# Autodesk Inventor assembly: Elevator Motor Assembly_MIR1 (nano)
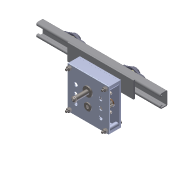
[picture p0: Inventor's stored thumbnail of the model, 180x180]
Saved by Autodesk Inventor 2015 (Build 190159000, 159)
## iProperties
Created: 2015-01-24
Part Number: Elevator Motor Assembly_MIR1 (nano)
Document SubType Name: Assembly
Designer: Peter
Author: Peter
## Documents named in this file (5)
- C:\Users\Tanner\Documents\GitHub\FIRST-Team-1719-CAD-Team\2015 Robot CAD\Lifter Super Structure\Tower\Elevator Motor Assembly\Elevator Motor Assembly_MIR1 (nano).iam
- C:\Users\Tanner\Documents\GitHub\FIRST-Team-1719-CAD-Team\2015 Robot CAD\Lifter Super Structure\Tower\Elevator Motor Assembly\Lower Motor Mount_MIR1.ipt
- C:\Users\Tanner\Documents\GitHub\FIRST-Team-1719-CAD-Team\2015 Robot CAD\Lifter Super Structure\Tower\Elevator Motor Assembly\Andy Mark Tough Box_MIR1.iam
- C:\Users\Tanner\Documents\GitHub\FIRST-Team-1719-CAD-Team\2015 Robot CAD\Lifter Super Structure\Tower\Elevator Motor Assembly\Horizontal-Unistrut-Tower-Connector-15_MIR1.ipt
- C:\Users\Tanner\Documents\GitHub\FIRST-Team-1719-CAD-Team\2015 Robot CAD\Lifter Super Structure\Tower\Elevator Motor Assembly\IGUS EF01-10\EFOI_10_1.iam
## Components (5 placed, 4 different names)
1. Lower Motor Mount_MIR1:1 — Mate:3, Mate:2, Mate:1, Mate:4, Flush:1
2. Andy Mark Tough Box_MIR1:1 [sub-assembly] — Mate:3, Mate:2, Mate:1
3. Horizontal-Unistrut-Tower-Connector-15_MIR1:1 — Mate:4, Flush:1, Mate:5, Mate:6, Tangent:1
4. EFOI_10_1:1 [sub-assembly] — Mate:5, Tangent:1
5. EFOI_10_1:2 [sub-assembly] — Mate:6
## Relationships (8: Mate 6, Flush 1, Tangent 1)
- Mate:3: Lower Motor Mount_MIR1:1 ↔ Andy Mark Tough Box_MIR1:1
- Mate:2: Lower Motor Mount_MIR1:1 ↔ Andy Mark Tough Box_MIR1:1
- Mate:1: Lower Motor Mount_MIR1:1 ↔ Andy Mark Tough Box_MIR1:1
- Mate:4: Lower Motor Mount_MIR1:1 ↔ Horizontal-Unistrut-Tower-Connector-15_MIR1:1
- Flush:1: Lower Motor Mount_MIR1:1 ↔ Horizontal-Unistrut-Tower-Connector-15_MIR1:1
- Mate:5: Horizontal-Unistrut-Tower-Connector-15_MIR1:1 ↔ EFOI_10_1:1
- Mate:6: Horizontal-Unistrut-Tower-Connector-15_MIR1:1 ↔ EFOI_10_1:2
- Tangent:1 (50.8 mm): Horizontal-Unistrut-Tower-Connector-15_MIR1:1 ↔ EFOI_10_1:1
